# Autodesk Inventor assembly: SAFRS-A-0006
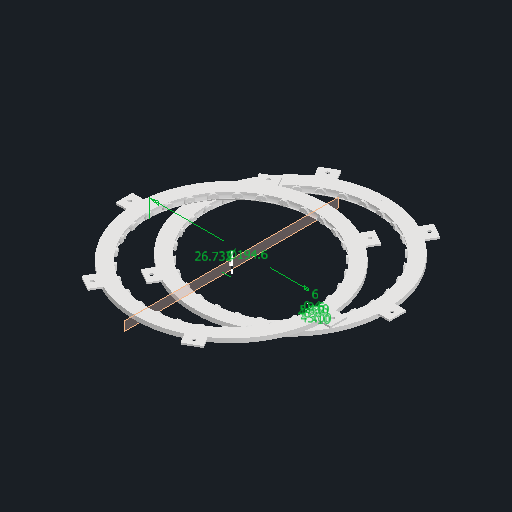
[picture p0: Inventor's stored thumbnail of the model, 512x512]
Saved by Autodesk Inventor 2026.2 (Build 302298000, 298)
## iProperties
Created: 2025-12-01
Part Number: SAFRS-A-0006
Document SubType Name: Assembly
Designer: jaewook
Author: jaewook
Title: Fixer Assembly
## Documents named in this file (4)
- C:\Users\jk000\OneDrive\Desktop\git\SAFRS\mechanical\inventor\02__subassemblies\fixer_assembly.iam
- C:\Users\jk000\OneDrive\Desktop\git\SAFRS\mechanical\inventor\01_parts\fixer_v1.ipt
- C:\Users\jk000\OneDrive\Desktop\git\SAFRS\mechanical\inventor\01_parts\fixer_left_v1.ipt
- C:\Users\jk000\OneDrive\Desktop\git\SAFRS\mechanical\inventor\01_parts\fixer_right_v1.ipt
## Components (3 placed, 3 different names)
1. fixer_v1:1
2. fixer_left_v1:1 — 메이트:1, 메이트:2, 메이트:3
3. fixer_right_v1:1 — 메이트:1, 메이트:2, 메이트:3
## Relationships (3: Mate 3)
- 메이트:1 [Mate]: fixer_left_v1:1 ↔ fixer_right_v1:1
- 메이트:2 [Mate]: fixer_left_v1:1 ↔ fixer_right_v1:1
- 메이트:3 [Mate]: fixer_left_v1:1 ↔ fixer_right_v1:1
